# Autodesk Inventor assembly: 24x34 Side Rail sub
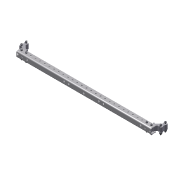
[picture p0: Inventor's stored thumbnail of the model, 180x180]
Saved by Autodesk Inventor 2013 (Build 170138000, 138)
## iProperties
Created: 2013-01-06
Part Number: 24x34 Side Rail sub
Document SubType Name: Assembly
Designer: Nemo
Author: Nemo
## Documents named in this file (4)
- H:\Nemo\Documents\Robotics\COTS Parts\Kit Frame\24x34 Side Rail sub.iam
- H:\Nemo\Documents\Robotics\COTS Parts\Kit Frame\CornerConnectAssyLeft.iam
- H:\Nemo\Documents\Robotics\COTS Parts\Kit Frame\CornerConnectAssyRight.iam
- H:\Nemo\Documents\Robotics\COTS Parts\Kit Frame\C Channel - Side 24x32.ipt
## Components (3 placed, 3 different names)
1. C Channel - Cut-01:1
2. CornerConnectAssyLeft:1 [sub-assembly]
3. CornerConnectAssyRight:1 [sub-assembly]
## Relationships (3: Mate 3)
- [Mate]: C Channel - Cut-01:1 ↔ CornerConnectAssyLeft:1
- [Mate]: C Channel - Cut-01:1 ↔ CornerConnectAssyLeft:1
- [Mate]: C Channel - Cut-01:1 ↔ CornerConnectAssyRight:1
